# Autodesk Inventor assembly: Chair
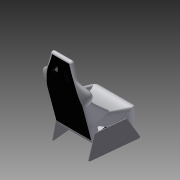
[picture p0: Inventor's stored thumbnail of the model, 180x180]
Saved by Autodesk Inventor 2015 (Build 190159000, 159)
## iProperties
Created: 2016-03-22
Part Number: Chair
Document SubType Name: Assembly
Designer: Mac
Author: Mac
## Documents named in this file (4)
- C:\Users\Mac\Desktop\MotionBase\CAD\MotionBaseCAD\Chair.iam
- C:\Users\Mac\Desktop\MotionBase\CAD\MotionBaseCAD\siege.ipt
- C:\Users\Mac\Desktop\MotionBase\CAD\MotionBaseCAD\Chair Support Side.ipt
- C:\Users\Mac\Desktop\MotionBase\CAD\MotionBaseCAD\Char Support Base.ipt
## Components (4 placed, 3 different names)
1. siege:1 — Mate:5, Mate:8
2. Chair Support Side:1 — Flush:1, Mate:3, Flush:2, Mate:6
3. Chair Support Side:2 — Mate:4, Flush:2, Mate:7
4. Char Support Base:1 — Flush:1, Mate:3, Mate:4, Mate:5
## Relationships (8: Mate 6, Flush 2)
- Flush:1 (-127 mm): Chair Support Side:1 ↔ Char Support Base:1
- Mate:3: Chair Support Side:1 ↔ Char Support Base:1
- Mate:4: Chair Support Side:2 ↔ Char Support Base:1
- Flush:2: Chair Support Side:1 ↔ Chair Support Side:2
- Mate:5: siege:1 ↔ Char Support Base:1
- Mate:6: Chair Support Side:1
- Mate:7: Chair Support Side:2
- Mate:8 (-355.6 mm): siege:1
